# Autodesk Inventor assembly: TankFlipper
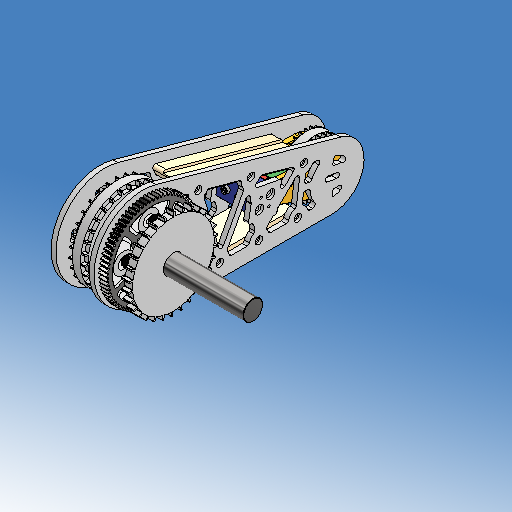
[picture p0: Inventor's stored thumbnail of the model, 512x512]
Saved by Autodesk Inventor 2025 (Build 290162000, 162)
## iProperties
Created: 2024-02-14
Part Number: TankFlipper
Document SubType Name: Assembly
Designer: seene
Author: seene
## Documents named in this file (9)
- C:\Users\seene\OneDrive\SBRT\Robocup Rescue\Drive\v1\TankFlipper Flipped.iam
- C:\Users\seene\OneDrive\SBRT\Robocup Rescue\Drive\v1\TANK flipper\panel_outside.ipt
- C:\Users\seene\OneDrive\SBRT\Robocup Rescue\Drive\v1\TANK flipper\panel_inside.ipt
- C:\Users\seene\OneDrive\SBRT\Robocup Rescue\Drive\v1\TANK flipper\flat chain guide.ipt
- C:\Users\seene\OneDrive\SBRT\Robocup Rescue\Drive\v1\TANK flipper\chain guide.ipt
- C:\Users\seene\OneDrive\SBRT\Robocup Rescue\Drive\v1\TANK flipper\TankFlipperAssembledDriveShaft.iam
- C:\Users\seene\OneDrive\SBRT\Robocup Rescue\Drive\v1\TANK flipper\flipper_tensioner _belt.iam
- C:\Users\seene\OneDrive\SBRT\Robocup Rescue\Drive\v1\TANK flipper\FlipperSpurGearMount.ipt
- C:\Users\seene\OneDrive\SBRT\Robocup Rescue\Drive\v1\TANK flipper\.25-20_FHCS_91263A553.ipt
## Components (12 placed, 8 different names)
1. panel_outside:1 — Mate:1, Mate:2, Mate:3, Mate:14, Mate:15, Mate:16
2. panel_inside:1 — Mate:4, Mate:5, Mate:6, Mate:9, Mate:10, Rigid:1, Mate:11, Mate:12, Mate:13
3. flat chain guide:1 — Mate:1, Mate:2, Mate:3, Mate:4, Mate:5, Mate:10
4. chain guide:1 — Mate:6, Mate:9
5. TankFlipperAssembledDriveShaft:1 [sub-assembly] — Rigid:1
6. flipper_tensioner _belt:1 [sub-assembly] — Mate:11, Mate:12, Mate:13
7. FlipperSpurGearMount:1 — Mate:14, Mate:15, Mate:16, Mate:17, Flush:1
8. .25-20_FHCS_91263A553:1 — Mate:17, Flush:1
9. .25-20_FHCS_91263A553:2
10. .25-20_FHCS_91263A553:3
11. .25-20_FHCS_91263A553:4
12. .25-20_FHCS_91263A553:5
## Component patterns: (5 elements, first: .25-20_FHCS_91263A553:1)
## Relationships (17: Mate 15, WeldJoint 1, Flush 1)
- Mate:1: panel_outside:1 ↔ flat chain guide:1
- Mate:2: panel_outside:1 ↔ flat chain guide:1
- Mate:3: panel_outside:1 ↔ flat chain guide:1
- Mate:4: panel_inside:1 ↔ flat chain guide:1
- Mate:5: panel_inside:1 ↔ flat chain guide:1
- Mate:6: panel_inside:1 ↔ chain guide:1
- Mate:9: panel_inside:1 ↔ chain guide:1
- Mate:10: panel_inside:1 ↔ flat chain guide:1
- Rigid:1 [WeldJoint]: panel_inside:1 ↔ TankFlipperAssembledDriveShaft:1
- Mate:11: panel_inside:1 ↔ flipper_tensioner _belt:1
- Mate:12: panel_inside:1 ↔ flipper_tensioner _belt:1
- Mate:13: panel_inside:1 ↔ flipper_tensioner _belt:1
- Mate:14: panel_outside:1 ↔ FlipperSpurGearMount:1
- Mate:15: panel_outside:1 ↔ FlipperSpurGearMount:1
- Mate:16: panel_outside:1 ↔ FlipperSpurGearMount:1
- Mate:17: FlipperSpurGearMount:1 ↔ .25-20_FHCS_91263A553:1
- Flush:1: FlipperSpurGearMount:1 ↔ .25-20_FHCS_91263A553:1
